# Autodesk Inventor assembly: TailCFDAssembly
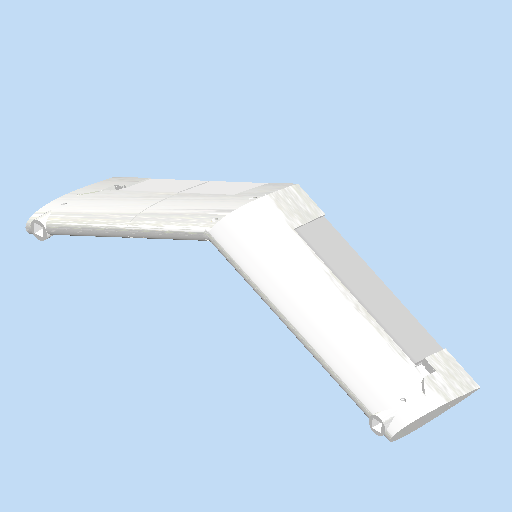
[picture p0: Inventor's stored thumbnail of the model, 512x512]
Saved by Autodesk Inventor 2026.1 (Build 301233000, 233)
## iProperties
Created: 2026-03-19
Part Number: TailCFDAssembly
Document SubType Name: Assembly
Designer: mateo
Author: mateo
## Documents named in this file (3)
- C:\GitHub\Senior-Design-UAV\Elytra CAD\CFD Assembly\TailCFDAssembly.iam
- C:\GitHub\Senior-Design-UAV\Elytra CAD\CFD Parts\TailCFD.ipt
- C:\GitHub\Senior-Design-UAV\Elytra CAD\CFD Parts\Vtail_MIR.ipt
## Components (3 placed, 2 different names)
1. TailCFD:1 — Mate:1, Mate:2, Mate:3, Insert:1, Insert:2
2. Vtail_MIR:1 — Insert:1
3. Vtail_MIR:2 — Insert:2
## Relationships (5: Mate 3, Insert 2)
- Mate:1: TailCFD:1
- Mate:2: TailCFD:1
- Mate:3: TailCFD:1
- Insert:1 (0.05 mm): TailCFD:1 ↔ Vtail_MIR:1
- Insert:2: TailCFD:1 ↔ Vtail_MIR:2
